# Autodesk Inventor assembly: tEST
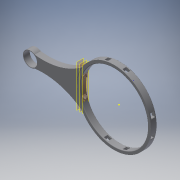
[picture p0: Inventor's stored thumbnail of the model, 180x180]
Saved by Autodesk Inventor 2017 (Build 210142000, 142)
## iProperties
Part Number: tEST
Material: Générique
Document SubType Name: Assembly
Designer: Thomas
Author: Thomas
## Documents named in this file (3)
- C:\Users\Thomas\Documents\Modele 3D\Drone\tEST.iam
- C:\Users\Thomas\Documents\Modele 3D\Drone\Aile.ipt
- C:\Users\Thomas\Documents\Modele 3D\Drone\Attache centre.ipt
## Components (2 placed, 2 different names)
1. Aile:1 — Affleurement:1, Placage:1
2. Attache centre:1 — Affleurement:1, Placage:1
## Relationships (2: Flush 1, Mate 1)
- Affleurement:1 [Flush]: Aile:1 ↔ Attache centre:1
- Placage:1 [Mate]: Aile:1 ↔ Attache centre:1
